# Autodesk Inventor assembly: Montagem KS D
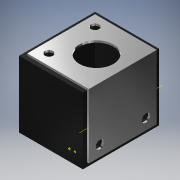
[picture p0: Inventor's stored thumbnail of the model, 180x180]
Saved by Autodesk Inventor 2019 (Build 230136000, 136)
## iProperties
Created: 2020-06-04
Part Number: Montagem KS D
Material: Genérico
Document SubType Name: Assembly
Designer: eliane
Author: eliane
## Documents named in this file (3)
- G:\Meu Drive\Projetos\Projeto 2020 2021\Eletrônica 2020-2021\Projeção mecânica\KS D\Montagem KS D.iam
- G:\Meu Drive\Projetos\Projeto 2020 2021\Eletrônica 2020-2021\Projeção mecânica\KS D\ks dianteiro F.ipt
- G:\Meu Drive\Projetos\Projeto 2020 2021\Eletrônica 2020-2021\Projeção mecânica\KS D\KS diant C.ipt
## Components (2 placed, 2 different names)
1. ks dianteiro F:1 — Alinhamento:1, Coincidência:1, Coincidência:2, Coincidência:3, Flush:2
2. KS diant C:1 — Alinhamento:1, Coincidência:1, Coincidência:2, Coincidência:3, Mate:4, Mate:5
## Relationships (7: Mate 5, Flush 2)
- Alinhamento:1 [Flush]: ks dianteiro F:1 ↔ KS diant C:1
- Coincidência:1 [Mate]: ks dianteiro F:1 ↔ KS diant C:1
- Coincidência:2 [Mate]: ks dianteiro F:1 ↔ KS diant C:1
- Coincidência:3 [Mate]: ks dianteiro F:1 ↔ KS diant C:1
- Mate:4: KS diant C:1
- Mate:5: KS diant C:1
- Flush:2 (12.7 mm): ks dianteiro F:1
